# Autodesk Inventor assembly: Złożenie
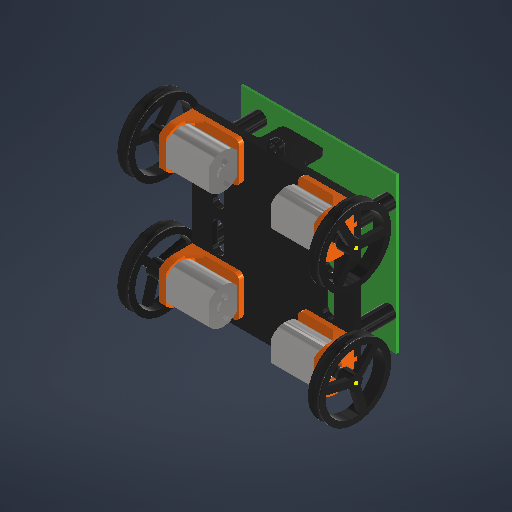
[picture p0: Inventor's stored thumbnail of the model, 512x512]
Saved by Autodesk Inventor 2026 (Build 300175000, 175)
## iProperties
Created: 2025-04-26
Part Number: Złożenie
Document SubType Name: Assembly
Designer: isan
Author: isan
## Documents named in this file (7)
- E:\Conan II enhanced\Złożenie.iam
- E:\Conan II enhanced\Podstawa.ipt
- E:\Conan II enhanced\Trzymak2.ipt
- E:\Conan II enhanced\Koło.ipt
- E:\Conan II enhanced\Silnik.ipt
- E:\Conan II enhanced\PCB.ipt
- E:\Conan II enhanced\Uchwyt.ipt
## Components (15 placed, 6 different names)
1. Podstawa:1 — Mate:1, Flush:1, Flush:2, Flush:3, Flush:4, Flush:5, Flush:6, Flush:7, Flush:8, Mate:21, Mate:22, Mate:23, Mate:24, Mate:25, Mate:26, Mate:27, Mate:32, Mate:33, Mate:37
2. Trzymak2:1 — Mate:1, Flush:1, Flush:2, Mate:14, Mate:15, Mate:16
3. Trzymak2:2 — Flush:3, Flush:4, Mate:11, Mate:12, Mate:13, Mate:26
4. Trzymak2:3 — Flush:7, Flush:8, Mate:5, Mate:6, Mate:7, Mate:25
5. Trzymak2:4 — Flush:5, Flush:6, Mate:8, Mate:9, Mate:10, Mate:27
6. Koło:1 — Mate:18, Mate:31
7. Koło:2 — Mate:17, Mate:29
8. Koło:3 — Mate:20, Mate:28
9. Koło:4 — Mate:19, Mate:30
10. Silnik:1 — Mate:11, Mate:12, Mate:13, Mate:18, Mate:31
11. Silnik:2 — Mate:5, Mate:6, Mate:7, Mate:20, Mate:28
12. Silnik:3 — Mate:8, Mate:9, Mate:10, Mate:17, Mate:29
13. Silnik:4 — Mate:14, Mate:15, Mate:16, Mate:19, Mate:30
14. PCB:1 — Mate:21, Mate:22, Mate:23, Mate:24
15. Uchwyt:1 — Mate:32, Mate:33, Mate:37
## Relationships (39: Mate 31, Flush 8)
- Mate:1: Podstawa:1 ↔ Trzymak2:1
- Flush:1: Podstawa:1 ↔ Trzymak2:1
- Flush:2: Podstawa:1 ↔ Trzymak2:1
- Flush:3: Podstawa:1 ↔ Trzymak2:2
- Flush:4: Podstawa:1 ↔ Trzymak2:2
- Flush:5: Podstawa:1 ↔ Trzymak2:4
- Flush:6: Podstawa:1 ↔ Trzymak2:4
- Flush:7: Podstawa:1 ↔ Trzymak2:3
- Flush:8: Podstawa:1 ↔ Trzymak2:3
- Mate:5: Trzymak2:3 ↔ Silnik:2
- Mate:6: Trzymak2:3 ↔ Silnik:2
- Mate:7: Trzymak2:3 ↔ Silnik:2
- Mate:8: Trzymak2:4 ↔ Silnik:3
- Mate:9: Trzymak2:4 ↔ Silnik:3
- Mate:10: Trzymak2:4 ↔ Silnik:3
- Mate:11: Trzymak2:2 ↔ Silnik:1
- Mate:12: Trzymak2:2 ↔ Silnik:1
- Mate:13: Trzymak2:2 ↔ Silnik:1
- Mate:14: Trzymak2:1 ↔ Silnik:4
- Mate:15: Trzymak2:1 ↔ Silnik:4
- Mate:16: Trzymak2:1 ↔ Silnik:4
- Mate:17: Koło:2 ↔ Silnik:3
- Mate:18: Koło:1 ↔ Silnik:1
- Mate:19: Koło:4 ↔ Silnik:4
- Mate:20: Koło:3 ↔ Silnik:2
- Mate:21: Podstawa:1 ↔ PCB:1
- Mate:22: Podstawa:1 ↔ PCB:1
- Mate:23: Podstawa:1 ↔ PCB:1
- Mate:24: Podstawa:1 ↔ PCB:1
- Mate:25: Podstawa:1 ↔ Trzymak2:3
- Mate:26: Podstawa:1 ↔ Trzymak2:2
- Mate:27: Podstawa:1 ↔ Trzymak2:4
- Mate:28: Koło:3 ↔ Silnik:2
- Mate:29: Koło:2 ↔ Silnik:3
- Mate:30: Koło:4 ↔ Silnik:4
- Mate:31: Koło:1 ↔ Silnik:1
- Mate:32: Podstawa:1 ↔ Uchwyt:1
- Mate:33: Podstawa:1 ↔ Uchwyt:1
- Mate:37: Podstawa:1 ↔ Uchwyt:1
